# Autodesk Inventor assembly: Talp
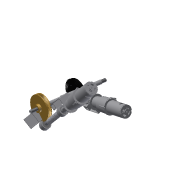
[picture p0: Inventor's stored thumbnail of the model, 180x180]
Saved by Autodesk Inventor 2015 SP1 (Build 190203100, 203)
## iProperties
Created: 2015-02-23
Part Number: Talp
Document SubType Name: Assembly
Designer: laca
Author: laca
## Documents named in this file (11)
- C:\Users\laca\Desktop\Allamvizsga\Invntor\RobotMechanikaForMAtlabVer2\Talp.iam
- C:\Users\laca\Desktop\Allamvizsga\Invntor\RobotMechanikaForMAtlabVer2\NagyTengely.ipt
- C:\Users\laca\Desktop\Allamvizsga\Invntor\RobotMechanikaForMAtlabVer2\SpanoloAnya.ipt
- C:\Users\laca\Desktop\Allamvizsga\Invntor\RobotMechanikaForMAtlabVer2\Tavolsagtarto.ipt
- C:\Users\laca\Desktop\Allamvizsga\Invntor\RobotMechanikaForMAtlabVer2\Worm Gear1.ipt
- C:\Users\laca\Desktop\Allamvizsga\Invntor\RobotMechanikaForMAtlabVer2\Bisztositek.ipt
- C:\Users\laca\Desktop\Allamvizsga\Invntor\RobotMechanikaForMAtlabVer2\Bevel Gears2.iam
- C:\Users\laca\Desktop\Allamvizsga\Invntor\RobotMechanikaForMAtlabVer2\MotorKerekHajtas.iam
- C:\Users\laca\Desktop\Allamvizsga\Invntor\RobotMechanikaForMAtlabVer2\MotorEsOrsoHajtas.iam
- C:\Users\laca\Desktop\Allamvizsga\Invntor\RobotMechanikaForMAtlabVer2\KarMerev.iam
- C:\Users\laca\Desktop\Allamvizsga\Invntor\RobotMechanikaForMAtlabVer2\InkrementalisFoliaEsNullAtmenet.iam
## Components (10 placed, 10 different names)
1. NagyTengely:1 — Insert:2, Cylindrical:8
2. SpanoloAnya:3 — Insert:2
3. Tavolsagtarto:1
4. Bisztositek:1 — Cylindrical:9, Angle:1, Mate:10
5. MotorEsOrsoHajtas:1 [sub-assembly]
6. Bevel Gears:1 [sub-assembly] — Flush:1, Insert:15
7. MotorKerekHajtas:1 [sub-assembly] — Flush:1, Insert:15
8. Worm Gear1:2 — Cylindrical:8, Cylindrical:9, Tangent:1
9. KarMerev:1 [sub-assembly]
10. InkrementalisFoliaEsNullAtmenet:1 [sub-assembly]
## Relationships (19: RevoluteJoint 4, CylindricalJoint 4, Mate 4, Insert 2, WeldJoint 1, RelateRotation 1, Angle 1, Tangent 1, Flush 1)
- [RevoluteJoint]: NagyTengely:1 ↔ KarMerev:1
- [RevoluteJoint]: Tavolsagtarto:1 ↔ KarMerev:1
- [WeldJoint] (-5 mm): NagyTengely:1 ↔ InkrementalisFoliaEsNullAtmenet:1
- [CylindricalJoint]: NagyTengely:1 ↔ Bisztositek:1
- [RevoluteJoint]: Bevel Gears:1 ↔ KarMerev:1
- [RevoluteJoint]: Bevel Gears:1 ↔ KarMerev:1
- [CylindricalJoint]: Bevel Gears:1 ↔ MotorKerekHajtas:1
- Insert:2: NagyTengely:1 ↔ SpanoloAnya:3
- [Mate]: MotorEsOrsoHajtas:1 ↔ Worm Gear1:2
- [Mate] (41.004 mm): MotorEsOrsoHajtas:1 ↔ Worm Gear1:2
- [RelateRotation] (66 ul): MotorEsOrsoHajtas:1 ↔ Worm Gear1:2
- Cylindrical:8: NagyTengely:1 ↔ Worm Gear1:2
- Cylindrical:9: Bisztositek:1 ↔ Worm Gear1:2
- [Mate]: Worm Gear1:2 ↔ InkrementalisFoliaEsNullAtmenet:1
- Angle:1 (0 deg): Bisztositek:1
- Tangent:1: Worm Gear1:2
- Mate:10: Bisztositek:1
- Flush:1: Bevel Gears:1 ↔ MotorKerekHajtas:1
- Insert:15: Bevel Gears:1 ↔ MotorKerekHajtas:1
## Named parameters: d31_d40 = 0 mm, d32_d41 = 54.124178 deg, d37_d38 = 0 mm, d38_d39 = 132.524149 deg
